# Autodesk Inventor assembly: Assembly
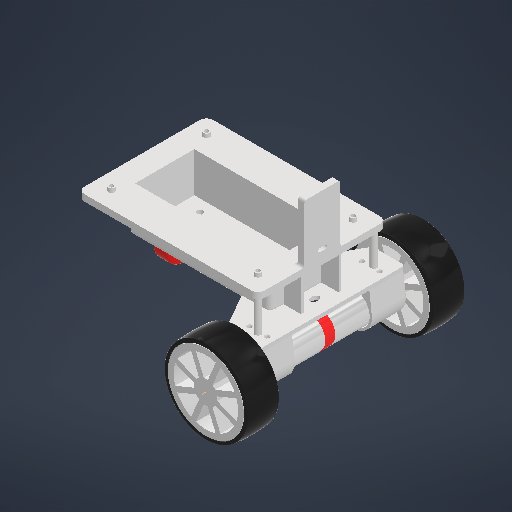
[picture p0: Inventor's stored thumbnail of the model, 512x512]
Saved by Autodesk Inventor 2027 (Build 310192000, 192)
## iProperties
Created: 2026-05-11
Part Number: Assembly
Document SubType Name: Assembly
Designer: maksi
Author: maksi
## Documents named in this file (6)
- C:\obsidian\main\mero\3d_parts\Assembly.iam
- C:\obsidian\main\mero\3d_parts\dc12v1200rpm.ipt
- C:\obsidian\main\mero\3d_parts\body.ipt
- C:\obsidian\main\mero\3d_parts\roller.ipt
- C:\obsidian\main\mero\3d_parts\wheel.ipt
- C:\obsidian\main\mero\3d_parts\motor_holder.ipt
## Components (8 placed, 5 different names)
1. dc12v1200rpm:1 — Rigid:2, Rotational:2
2. body:1 — Rigid:3, Rigid:4, Rigid:5, Mate:1, Flush:1, Flush:2
3. dc12v1200rpm:2 — Rigid:1, Rotational:1
4. roller:1 — Rigid:5
5. wheel:1 — Rotational:2
6. wheel:2 — Rotational:1
7. motor_holder:1 — Rigid:2, Rigid:4
8. motor_holder:2 — Rigid:1, Rigid:3
## Relationships (10: WeldJoint 5, RevoluteJoint 2, Flush 2, Mate 1)
- Rigid:1 [WeldJoint]: dc12v1200rpm:2 ↔ motor_holder:2
- Rigid:2 [WeldJoint]: dc12v1200rpm:1 ↔ motor_holder:1
- Rotational:1 [RevoluteJoint] (-2 mm): dc12v1200rpm:2 ↔ wheel:2
- Rotational:2 [RevoluteJoint] (-2 mm): dc12v1200rpm:1 ↔ wheel:1
- Rigid:3 [WeldJoint]: body:1 ↔ motor_holder:2
- Rigid:4 [WeldJoint]: body:1 ↔ motor_holder:1
- Rigid:5 [WeldJoint]: body:1 ↔ roller:1
- Mate:1: body:1
- Flush:1: body:1
- Flush:2: body:1
